# Autodesk Inventor assembly: 90 Barcket
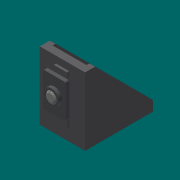
[picture p0: Inventor's stored thumbnail of the model, 180x180]
Saved by Autodesk Inventor 2016 (Build 200138000, 138)
## iProperties
Created: 2015-06-02
Part Number: 90 Barcket
Document SubType Name: Assembly
Designer: Sawaiz Syed
Author: Sawaiz Syed
## Documents named in this file (4)
- C:\Users\Sawaiz\Documents\data\projects\cncBlackBox\frame\90 Barcket.iam
- C:\Users\Sawaiz\Documents\data\projects\cncBlackBox\frame\HBLFSN5.ipt
- C:\Users\Sawaiz\Documents\data\projects\cncBlackBox\hardware\m5x10.ipt
- C:\Users\Sawaiz\Documents\data\projects\cncBlackBox\hardware\m5TNut.ipt
## Components (5 placed, 3 different names)
1. HBLFSN5:1 — Mate:9, Angle:2, Mate:11, Angle:3, Mate:12, Mate:13, Mate:14, Mate:15
2. m5x10:1 — Mate:12, Mate:14, Mate:16
3. m5x10:2 — Mate:13, Mate:15, Mate:17
4. m5TNut:1 — Mate:9, Angle:2, Mate:16
5. m5TNut:2 — Mate:11, Angle:3, Mate:17
## Relationships (10: Mate 8, Angle 2)
- Mate:9 (2 mm): HBLFSN5:1 ↔ m5TNut:1
- Angle:2 (0 deg): HBLFSN5:1 ↔ m5TNut:1
- Mate:11 (2 mm): HBLFSN5:1 ↔ m5TNut:2
- Angle:3 (0 deg): HBLFSN5:1 ↔ m5TNut:2
- Mate:12: HBLFSN5:1 ↔ m5x10:1
- Mate:13: HBLFSN5:1 ↔ m5x10:2
- Mate:14: HBLFSN5:1 ↔ m5x10:1
- Mate:15: HBLFSN5:1 ↔ m5x10:2
- Mate:16: m5x10:1 ↔ m5TNut:1
- Mate:17: m5x10:2 ↔ m5TNut:2
